# Autodesk Inventor assembly: Funnel Assembly
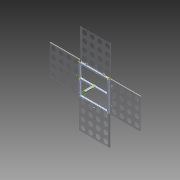
[picture p0: Inventor's stored thumbnail of the model, 180x180]
Saved by Autodesk Inventor 2014 (Build 180170000, 170)
## iProperties
Created: 2014-01-05
Part Number: Funnel Assembly
Document SubType Name: Assembly
Designer: Michael
Mass: 2573.42 g
Surface Area: 24754.3 cm^2
Volume: 1179.23 cm^3
Density: 2.1823 g/cm^3
Author: Michael
## Documents named in this file (3)
- C:\Users\Michael\Documents\Robotics\2014 Season\Funnel Catcher\Funnel Assembly.iam
- C:\Users\Michael\Documents\Robotics\2014 Season\Funnel Catcher\Funnel Plate Assembly.iam
- C:\Users\Michael\Documents\Robotics\2014 Season\Funnel Catcher\Back Funnel Frame.iam
## Components (5 placed, 2 different names)
1. Funnel Plate Assembly:1 [sub-assembly] — Insert:9, Insert:10
2. Funnel Plate Assembly:3 [sub-assembly] — Insert:5, Insert:6
3. Funnel Plate Assembly:4 [sub-assembly] — Insert:11, Insert:12
4. Funnel Plate Assembly:5 [sub-assembly] — Insert:7, Insert:8
5. Back Funnel Frame:1 [sub-assembly] — Insert:5, Insert:6, Insert:7, Insert:8, Insert:9, Insert:10, Insert:11, Insert:12
## Relationships (8: Insert 8)
- Insert:5: Funnel Plate Assembly:3 ↔ Back Funnel Frame:1
- Insert:6: Funnel Plate Assembly:3 ↔ Back Funnel Frame:1
- Insert:7: Funnel Plate Assembly:5 ↔ Back Funnel Frame:1
- Insert:8: Funnel Plate Assembly:5 ↔ Back Funnel Frame:1
- Insert:9: Funnel Plate Assembly:1 ↔ Back Funnel Frame:1
- Insert:10: Funnel Plate Assembly:1 ↔ Back Funnel Frame:1
- Insert:11: Funnel Plate Assembly:4 ↔ Back Funnel Frame:1
- Insert:12: Funnel Plate Assembly:4 ↔ Back Funnel Frame:1
